# Autodesk Inventor assembly: Ensamble IAM
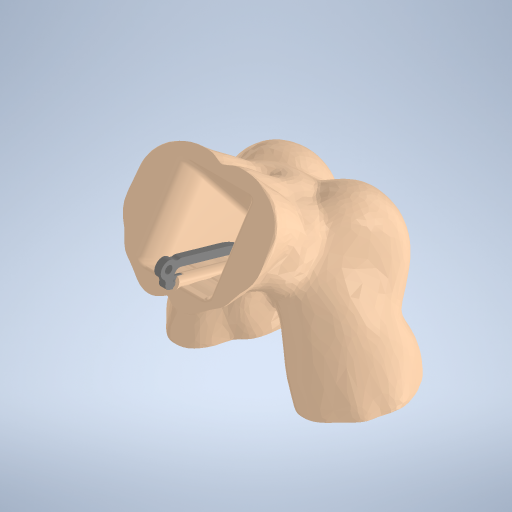
[picture p0: Inventor's stored thumbnail of the model, 512x512]
Saved by Autodesk Inventor 2024 (Build 280153000, 153)
## iProperties
Created: 2023-08-24
Part Number: Ensamble IAM
Document SubType Name: Assembly
Designer: gdpg
Author: gdpg
## Documents named in this file (3)
- C:\Users\gdpg\Desktop\MANIQUI\MODELO FINAL\Ensamble IAM.iam
- C:\Users\gdpg\Desktop\MANIQUI\MODELO FINAL\Maniqui completo.ipt
- C:\Users\gdpg\Desktop\MANIQUI\MODELO FINAL\Tubo de prostata.ipt
## Components (2 placed, 2 different names)
1. Maniqui completo:1 — Insertar:1
2. Tubo de prostata:1 — Insertar:1
## Relationships (1: Insert 1)
- Insertar:1 (30 mm): Maniqui completo:1 ↔ Tubo de prostata:1
